# Autodesk Inventor assembly: ASY MSC 089 gills base
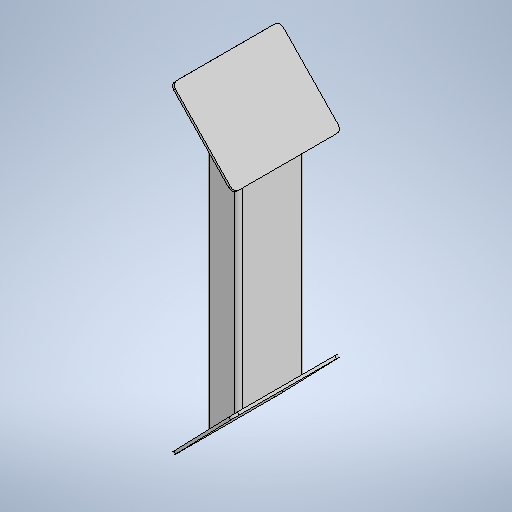
[picture p0: Inventor's stored thumbnail of the model, 512x512]
Saved by Autodesk Inventor 2025 (Build 290162010, 162A)
## iProperties
Created: 2024-09-02
Part Number: ASY MSC 089 gills base
Document SubType Name: Assembly
Designer: admin
Author: admin
## Documents named in this file (3)
- C:\Users\user\YandexDisk\домашниий пк\Inventor\Manturovo\Manturovo_Se-clar\ASY MSC 089 gills base.iam
- C:\Users\user\YandexDisk\домашниий пк\Inventor\Manturovo\Manturovo_Se-clar\MSC 085 bottom support gills.ipt
- C:\Users\user\YandexDisk\домашниий пк\Inventor\Manturovo\Manturovo_Se-clar\MSC 087 bottom plate gills.ipt
## Components (3 placed, 2 different names)
1. MSC 085 bottom support gills:1
2. MSC 087 bottom plate gills:2
3. MSC 087 bottom plate gills:1
## Relationships (2: WeldJoint 2)
- [WeldJoint]: MSC 085 bottom support gills:1 ↔ MSC 087 bottom plate gills:1
- [WeldJoint]: MSC 085 bottom support gills:1 ↔ MSC 087 bottom plate gills:2
